# Autodesk Inventor assembly: chwytak
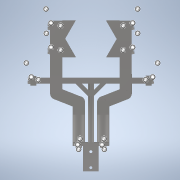
[picture p0: Inventor's stored thumbnail of the model, 180x180]
Saved by Autodesk Inventor 2022.1 (Build 261234020, 234B)
## iProperties
Created: 2022-05-02
Part Number: chwytak
Document SubType Name: Assembly
Designer: Kacper Kaczmarski
Mass: 211.841 g
Surface Area: 230.221 cm^2
Volume: 27.3344 cm^3
Density: 7.75 g/cm^3
Author: Kacper Kaczmarski
## Documents named in this file (18)
- D:\Studia\Studia\S2\3DCNC\chwytak\chwytak.iam
- D:\Studia\Studia\S2\3DCNC\chwytak\adapter.ipt
- D:\Studia\Studia\S2\3DCNC\chwytak\Część L5.ipt
- D:\Studia\Studia\S2\3DCNC\chwytak\Część L1.ipt
- D:\Studia\Studia\S2\3DCNC\chwytak\ramie.ipt
- C:\Users\Kacper\Documents\Inventor\Content Center Files\R2022\pl-PL\ISO 1207(2)\ISO 1207 - M3 x 8.ipt
- D:\Studia\Studia\S2\3DCNC\chwytak\część L3.ipt
- D:\Studia\Studia\S2\3DCNC\chwytak\zatyczka na szyne.ipt
- D:\Studia\Studia\S2\3DCNC\chwytak\szczęka.ipt
- D:\Studia\Studia\S2\3DCNC\chwytak\sworzeń.ipt
- C:\Users\Kacper\Documents\Inventor\Content Center Files\R2022\pl-PL\ISO 1207(2)\ISO 1207 - M3 x 10.ipt
- C:\Users\Kacper\Documents\Inventor\Content Center Files\R2022\pl-PL\ISO 1207(2)\ISO 1207 - M3 x 14.ipt
- D:\Studia\Studia\S2\3DCNC\chwytak\chwytak\AIP\FEA\dyk7d49cw.fins
- D:\Studia\Studia\S2\3DCNC\chwytak\chwytak\AIP\FEA\dyk7d49ds.fsat
- D:\Studia\Studia\S2\3DCNC\chwytak\chwytak\AIP\FEA\dyk7d49ds.ftes
- D:\Studia\Studia\S2\3DCNC\chwytak\chwytak\AIP\FEA\dyk7d49ds.fwiz
- D:\Studia\Studia\S2\3DCNC\chwytak\chwytak\AIP\FEA\dyk7d49hc.fmsh
- D:\Studia\Studia\S2\3DCNC\chwytak\chwytak\AIP\FEA\dyk7d49hd.fres
## Components (24 placed, 11 different names)
1. adapter:1 — Zestawiające:1, Zestawiające:2, Zestawiające:3, Zestawiające:4, Zestawiające:5, Zestawiające:6, Zestawiające:7, Zestawiające:14, Równoległe:1, Zestawiające:49
2. Część L5:1 — Zestawiające:2, Zestawiające:10, Zestawiające:12, Zestawiające:14, Zestawiające:23, Zestawiające:48
3. Część L5:2 — Zestawiające:1, Zestawiające:17, Zestawiające:20, Zestawiające:24, Zestawiające:47, Zestawiające:49
4. Część L1:1 — Zestawiające:7, Zestawiające:8, Zestawiające:9, Równoległe:1, Zestawiające:21, Zestawiające:22, Zestawiające:26, Zestawiające:27, Zestawiające:30, Zestawiające:31
5. ramie:1 — Zestawiające:18, Zestawiające:19, Zestawiające:21, Zestawiające:22, Zestawiające:25, Zestawiające:34, Zestawiające:35, Równoległe:2, Zestawiające:38, Zestawiające:39, Zestawiające:40, Zestawiające:41, Zestawiające:46
6. ramie:2 — Zestawiające:8, Zestawiające:9, Zestawiające:11, Zestawiające:13, Zestawiające:36, Zestawiające:37, Równoległe:3, Zestawiające:42, Zestawiające:43, Zestawiające:44, Zestawiające:45, Zestawiające:50
7. ISO 1207 M3 x 8:1 — Zestawiające:3, Zestawiające:4
8. ISO 1207 M3 x 8:2 — Zestawiające:5, Zestawiające:6
9. część L3:1 — Zestawiające:17, Zestawiające:18, Zestawiające:19, Zestawiające:20
10. część L3:2 — Zestawiające:10, Zestawiające:11, Zestawiające:23
11. zatyczka na szyne:1 — Zestawiające:30, Zestawiające:31, Zestawiające:32, Zestawiające:33
12. zatyczka na szyne:2 — Zestawiające:26, Zestawiające:27, Zestawiające:28, Zestawiające:29
13. szczęka:1 — Zestawiające:36, Zestawiające:37, Równoległe:3
14. szczęka:2 — Zestawiające:34, Zestawiające:35, Równoległe:2
15. sworzeń:1 — Zestawiające:13, Zestawiające:50
16. sworzeń:2 — Zestawiające:12, Zestawiające:48
17. sworzeń:3 — Zestawiające:24, Zestawiające:47
18. sworzeń:4 — Zestawiające:25, Zestawiające:46
19. ISO 1207 M3 x 10:1 — Zestawiające:28, Zestawiające:29
20. ISO 1207 M3 x 10:2 — Zestawiające:32, Zestawiające:33
21. ISO 1207 M3 x 14:1 — Zestawiające:38, Zestawiające:39
22. ISO 1207 M3 x 14:2 — Zestawiające:40, Zestawiające:41
23. ISO 1207 M3 x 14:3 — Zestawiające:42, Zestawiające:43
24. ISO 1207 M3 x 14:4 — Zestawiające:44, Zestawiające:45
## Relationships (51: Mate 48, Flush 3)
- Zestawiające:1 [Mate]: adapter:1 ↔ Część L5:2
- Zestawiające:2 [Mate]: adapter:1 ↔ Część L5:1
- Zestawiające:3 [Mate]: adapter:1 ↔ ISO 1207 M3 x 8:1
- Zestawiające:4 [Mate]: adapter:1 ↔ ISO 1207 M3 x 8:1
- Zestawiające:5 [Mate]: adapter:1 ↔ ISO 1207 M3 x 8:2
- Zestawiające:6 [Mate]: adapter:1 ↔ ISO 1207 M3 x 8:2
- Zestawiające:7 [Mate]: adapter:1 ↔ Część L1:1
- Zestawiające:8 [Mate]: Część L1:1 ↔ ramie:2
- Zestawiające:9 [Mate]: Część L1:1 ↔ ramie:2
- Zestawiające:10 [Mate]: Część L5:1 ↔ część L3:2
- Zestawiające:11 [Mate]: ramie:2 ↔ część L3:2
- Zestawiające:12 [Mate]: Część L5:1 ↔ sworzeń:2
- Zestawiające:13 [Mate]: ramie:2 ↔ sworzeń:1
- Zestawiające:14 [Mate]: adapter:1 ↔ Część L5:1
- Równoległe:1 [Flush]: adapter:1 ↔ Część L1:1
- Zestawiające:17 [Mate]: Część L5:2 ↔ część L3:1
- Zestawiające:18 [Mate]: ramie:1 ↔ część L3:1
- Zestawiające:19 [Mate]: ramie:1 ↔ część L3:1
- Zestawiające:20 [Mate]: Część L5:2 ↔ część L3:1
- Zestawiające:21 [Mate]: Część L1:1 ↔ ramie:1
- Zestawiające:22 [Mate]: Część L1:1 ↔ ramie:1
- Zestawiające:23 [Mate]: Część L5:1 ↔ część L3:2
- Zestawiające:24 [Mate]: Część L5:2 ↔ sworzeń:3
- Zestawiające:25 [Mate]: ramie:1 ↔ sworzeń:4
- Zestawiające:26 [Mate]: Część L1:1 ↔ zatyczka na szyne:2
- Zestawiające:27 [Mate]: Część L1:1 ↔ zatyczka na szyne:2
- Zestawiające:28 [Mate]: zatyczka na szyne:2 ↔ ISO 1207 M3 x 10:1
- Zestawiające:29 [Mate]: zatyczka na szyne:2 ↔ ISO 1207 M3 x 10:1
- Zestawiające:30 [Mate]: Część L1:1 ↔ zatyczka na szyne:1
- Zestawiające:31 [Mate]: Część L1:1 ↔ zatyczka na szyne:1
- Zestawiające:32 [Mate]: zatyczka na szyne:1 ↔ ISO 1207 M3 x 10:2
- Zestawiające:33 [Mate]: zatyczka na szyne:1 ↔ ISO 1207 M3 x 10:2
- Zestawiające:34 [Mate]: ramie:1 ↔ szczęka:2
- Zestawiające:35 [Mate]: ramie:1 ↔ szczęka:2
- Równoległe:2 [Flush]: ramie:1 ↔ szczęka:2
- Zestawiające:36 [Mate]: ramie:2 ↔ szczęka:1
- Zestawiające:37 [Mate]: ramie:2 ↔ szczęka:1
- Równoległe:3 [Flush]: ramie:2 ↔ szczęka:1
- Zestawiające:38 [Mate]: ramie:1 ↔ ISO 1207 M3 x 14:1
- Zestawiające:39 [Mate]: ramie:1 ↔ ISO 1207 M3 x 14:1
- Zestawiające:40 [Mate]: ramie:1 ↔ ISO 1207 M3 x 14:2
- Zestawiające:41 [Mate]: ramie:1 ↔ ISO 1207 M3 x 14:2
- Zestawiające:42 [Mate]: ramie:2 ↔ ISO 1207 M3 x 14:3
- Zestawiające:43 [Mate]: ramie:2 ↔ ISO 1207 M3 x 14:3
- Zestawiające:44 [Mate]: ramie:2 ↔ ISO 1207 M3 x 14:4
- Zestawiające:45 [Mate]: ramie:2 ↔ ISO 1207 M3 x 14:4
- Zestawiające:46 [Mate]: ramie:1 ↔ sworzeń:4
- Zestawiające:47 [Mate]: Część L5:2 ↔ sworzeń:3
- Zestawiające:48 [Mate]: Część L5:1 ↔ sworzeń:2
- Zestawiające:49 [Mate]: adapter:1 ↔ Część L5:2
- Zestawiające:50 [Mate]: ramie:2 ↔ sworzeń:1
## Named parameters: sa_0 = 1100, sa_1 = 1100
note: some values were not read from the file. Shown as the stored number, unit unknown: "sa_0", "sa_1".
